# Autodesk Inventor assembly: AS-00000002
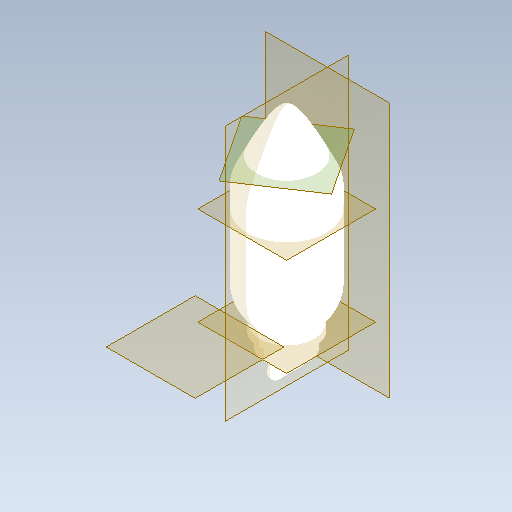
[picture p0: Inventor's stored thumbnail of the model, 512x512]
Saved by Autodesk Inventor 2020.1 (Build 241239000, 239)
## iProperties
Created: 2020-09-09
Part Number: AS-00000002
Document SubType Name: Assembly
Designer: Haynie R&D
Author: Haynie R&D
## Documents named in this file (3)
- C:\Users\hrd\Documents\Vault\Haynie Research\Designs\R&D\Telemetry\Nose Cone\Nose Cone.iam
- C:\Users\hrd\Documents\Vault\Haynie Research\Designs\R&D\Telemetry\Nose Cone\noze-cone-bottom.ipt
- C:\Users\hrd\Documents\Vault\Haynie Research\Designs\R&D\Telemetry\Nose Cone\noze-cone-top.ipt
## Components (2 placed, 2 different names)
1. noze-cone-top:1 — Mate:1, Mate:2, Mate:3, Flush:1, Flush:2
2. noze-cone-bottom:1 — Mate:1, Mate:2, Mate:4
## Relationships (6: Mate 4, Flush 2)
- Mate:1: noze-cone-top:1 ↔ noze-cone-bottom:1
- Mate:2: noze-cone-top:1 ↔ noze-cone-bottom:1
- Mate:3: noze-cone-top:1
- Mate:4: noze-cone-bottom:1
- Flush:1: noze-cone-top:1
- Flush:2 (-29 mm): noze-cone-top:1
